# Autodesk Inventor assembly: CIM Assembly
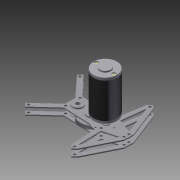
[picture p0: Inventor's stored thumbnail of the model, 180x180]
Saved by Autodesk Inventor 2013 (Build 170138000, 138)
## iProperties
Created: 2013-01-17
Part Number: CIM Assembly
Document SubType Name: Assembly
Designer: actoennies
Mass: 1104.36 g
Surface Area: 1234.15 cm^2
Volume: 493.223 cm^3
Density: 2.23906 g/cm^3
Author: actoennies
## Documents named in this file (9)
- \\NNHSSRV2.hs.sd203.org\ACToennies$\Robotics\Shooter\CIM Assembly.iam
- \\NNHSSRV2.hs.sd203.org\ACToennies$\Robotics\Shooter\CIM Bearing.ipt
- \\NNHSSRV2.hs.sd203.org\ACToennies$\Robotics\Shooter\Bearing.ipt
- \\NNHSSRV2.hs.sd203.org\ACToennies$\Robotics\Shooter\Bearing Plate.ipt
- \\NNHSSRV2.hs.sd203.org\ACToennies$\Robotics\Shooter\Hex Gear.ipt
- \\NNHSSRV2.hs.sd203.org\ACToennies$\Robotics\Shooter\Big Gear.ipt
- \\NNHSSRV2.hs.sd203.org\ACToennies$\Robotics\Parts\CIM Motor\Motors_FR801-001.iam
- \\NNHSSRV2.hs.sd203.org\ACToennies$\Robotics\Shooter\CIM Gear.ipt
- \\NNHSSRV2.hs.sd203.org\ACToennies$\Robotics\Shooter\Short Hex Shaft.ipt
## Components (13 placed, 8 different names)
1. CIM Bearing:1 — Insert:2, Insert:12
2. CIM Bearing:2 — Insert:1, Rotation:1, Rotation:2, Rotation:3
3. Bearing:1 — Flush:3, Flush:4, Mate:2, Insert:8
4. Bearing:2 — Insert:3, Mate:1, Flush:1, Flush:2
5. Bearing Plate:1 — Insert:1, Insert:3, Flush:7, Insert:10
6. Bearing Plate:2 — Insert:2, Insert:8, Flush:7, Insert:9, Mate:5, Mate:6
7. Hex Gear:1 — Mate:1, Flush:1, Flush:2, Flush:3, Flush:4, Mate:2
8. Big Gear:1 — Flush:8, Flush:9, Insert:11, Flush:10
9. Motors_FR801-001:1 [sub-assembly] — Rotation:1, Rotation:4, Rotation:6, Mate:5, Flush:12, Mate:6
10. CIM Gear:1 — Insert:12, Flush:12
11. Bearing:3 — Insert:9, Flush:8, Flush:9, Insert:11
12. Bearing:4 — Insert:10, Flush:10, Flush:11, Mate:3, Mate:4, Rotation:2, Rotation:3
13. Short Hex Shaft:1 — Flush:11, Mate:3, Mate:4, Rotation:4, Rotation:6
## Relationships (29: Flush 10, Insert 8, Mate 6, RelateRotation 5)
- Insert:1: CIM Bearing:2 ↔ Bearing Plate:1
- Insert:2: CIM Bearing:1 ↔ Bearing Plate:2
- Insert:3: Bearing:2 ↔ Bearing Plate:1
- Mate:1: Bearing:2 ↔ Hex Gear:1
- Flush:1: Bearing:2 ↔ Hex Gear:1
- Flush:2: Bearing:2 ↔ Hex Gear:1
- Flush:3: Bearing:1 ↔ Hex Gear:1
- Flush:4: Bearing:1 ↔ Hex Gear:1
- Mate:2: Bearing:1 ↔ Hex Gear:1
- Insert:8: Bearing:1 ↔ Bearing Plate:2
- Flush:7: Bearing Plate:1 ↔ Bearing Plate:2
- Insert:9: Bearing Plate:2 ↔ Bearing:3
- Insert:10: Bearing Plate:1 ↔ Bearing:4
- Flush:8: Big Gear:1 ↔ Bearing:3
- Flush:9: Big Gear:1 ↔ Bearing:3
- Insert:11: Big Gear:1 ↔ Bearing:3
- Insert:12: CIM Bearing:1 ↔ CIM Gear:1
- Flush:10: Big Gear:1 ↔ Bearing:4
- Flush:11: Bearing:4 ↔ Short Hex Shaft:1
- Mate:3: Bearing:4 ↔ Short Hex Shaft:1
- Mate:4: Bearing:4 ↔ Short Hex Shaft:1
- Rotation:1 [RelateRotation] (1 ul): CIM Bearing:2 ↔ Motors_FR801-001:1
- Rotation:2 [RelateRotation] (3.4286 ul): CIM Bearing:2 ↔ Bearing:4
- Rotation:3 [RelateRotation] (3.4286 ul): CIM Bearing:2 ↔ Bearing:4
- Rotation:4 [RelateRotation] (0.2917 ul): Motors_FR801-001:1 ↔ Short Hex Shaft:1
- Rotation:6 [RelateRotation] (0.2917 ul): Motors_FR801-001:1 ↔ Short Hex Shaft:1
- Mate:5: Bearing Plate:2 ↔ Motors_FR801-001:1
- Flush:12: Motors_FR801-001:1 ↔ CIM Gear:1
- Mate:6: Bearing Plate:2 ↔ Motors_FR801-001:1
